# Autodesk Inventor assembly: Intake&Outake
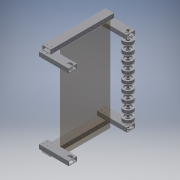
[picture p0: Inventor's stored thumbnail of the model, 180x180]
Saved by Autodesk Inventor 2018 (Build 220112000, 112)
## iProperties
Created: 2018-09-06
Part Number: Intake&Outake
Document SubType Name: Assembly
Designer: baoan
Author: baoan
## Documents named in this file (7)
- C:\Users\baoan\Documents\Inventor\Bunnybots\Intake&Outake\Intake&Outake.iam
- C:\Users\baoan\Documents\Inventor\Bunnybots\Intake&Outake\Vertical_intake_frame.ipt
- C:\Users\baoan\Documents\Inventor\Bunnybots\Intake&Outake\Horizontal_intake_hanger.ipt
- C:\Users\baoan\Documents\Inventor\Bunnybots\Intake&Outake\Bearing.ipt
- C:\Users\baoan\Documents\Inventor\Bunnybots\Intake&Outake\Hex_shaft.ipt
- C:\Users\baoan\Documents\Inventor\Bunnybots\Intake&Outake\36t_x_15mm_Wide_Aluminum_Pulley_HTD_5mm_1_2_Hex_217-4103.ipt
- C:\Users\baoan\Documents\Inventor\Bunnybots\Intake&Outake\Intake_backboard.ipt
## Components (21 placed, 6 different names)
1. Vertical_intake_frame:1 — Flush:1, Mate:1, Flush:2, Flush:5, Flush:6, Mate:3, Mate:19, Flush:14, Flush:16, Mate:20, Flush:17
2. Horizontal_intake_hanger:1 — Flush:1, Mate:1, Flush:2, Insert:7, Insert:8, Mate:21
3. Vertical_intake_frame:2 — Mate:2, Flush:3, Flush:4, Flush:5, Flush:6, Mate:3, Mate:17, Flush:13
4. Horizontal_intake_hanger:2 — Mate:2, Flush:3, Flush:4, Insert:5, Insert:6, Flush:12, Mate:16
5. Bearing:5 — Insert:6, Mate:14
6. Bearing:6 — Insert:5
7. Bearing:7 — Insert:7
8. Bearing:8 — Insert:8
9. Hex_shaft:2 — Flush:12, Angle:1
10. Horizontal_intake_hanger:3 — Mate:17, Flush:13, Flush:15
11. Horizontal_intake_hanger:4 — Mate:19, Flush:14, Flush:15, Flush:16
12. Intake_backboard:1 — Mate:20, Flush:17, Mate:21
13. 36t_x_15mm_Wide_Aluminum_Pulley_HTD_5mm_1_2_Hex_217-4103:1 — Mate:14, Angle:1, Mate:16
14. 36t_x_15mm_Wide_Aluminum_Pulley_HTD_5mm_1_2_Hex_217-4103:2
15. 36t_x_15mm_Wide_Aluminum_Pulley_HTD_5mm_1_2_Hex_217-4103:3
16. 36t_x_15mm_Wide_Aluminum_Pulley_HTD_5mm_1_2_Hex_217-4103:4
17. 36t_x_15mm_Wide_Aluminum_Pulley_HTD_5mm_1_2_Hex_217-4103:5
18. 36t_x_15mm_Wide_Aluminum_Pulley_HTD_5mm_1_2_Hex_217-4103:6
19. 36t_x_15mm_Wide_Aluminum_Pulley_HTD_5mm_1_2_Hex_217-4103:7
20. 36t_x_15mm_Wide_Aluminum_Pulley_HTD_5mm_1_2_Hex_217-4103:8
21. 36t_x_15mm_Wide_Aluminum_Pulley_HTD_5mm_1_2_Hex_217-4103:9
## Component patterns: (9 elements, first: 36t_x_15mm_Wide_Aluminum_Pulley_HTD_5mm_1_2_Hex_217-4103:1)
## Relationships (30: Flush 14, Mate 11, Insert 4, Angle 1)
- Flush:1: Vertical_intake_frame:1 ↔ Horizontal_intake_hanger:1
- Mate:1: Vertical_intake_frame:1 ↔ Horizontal_intake_hanger:1
- Flush:2: Vertical_intake_frame:1 ↔ Horizontal_intake_hanger:1
- Mate:2: Vertical_intake_frame:2 ↔ Horizontal_intake_hanger:2
- Flush:3: Vertical_intake_frame:2 ↔ Horizontal_intake_hanger:2
- Flush:4: Vertical_intake_frame:2 ↔ Horizontal_intake_hanger:2
- Flush:5: Vertical_intake_frame:1 ↔ Vertical_intake_frame:2
- Flush:6: Vertical_intake_frame:1 ↔ Vertical_intake_frame:2
- Mate:3 (508 mm): Vertical_intake_frame:1 ↔ Vertical_intake_frame:2
- [Flush]: Bearing:5 ↔ Bearing:6
- [Flush]: Bearing:7 ↔ Bearing:8
- [Mate]: Bearing:6 ↔ Hex_shaft:2
- [Mate]: Bearing:6 ↔ Hex_shaft:2
- Insert:5: Horizontal_intake_hanger:2 ↔ Bearing:6
- Insert:6: Horizontal_intake_hanger:2 ↔ Bearing:5
- Insert:7: Horizontal_intake_hanger:1 ↔ Bearing:7
- Insert:8: Horizontal_intake_hanger:1 ↔ Bearing:8
- Flush:12 (-12.7 mm): Horizontal_intake_hanger:2 ↔ Hex_shaft:2
- Mate:14: Bearing:5 ↔ 36t_x_15mm_Wide_Aluminum_Pulley_HTD_5mm_1_2_Hex_217-4103:1
- Angle:1 (0 deg): Hex_shaft:2 ↔ 36t_x_15mm_Wide_Aluminum_Pulley_HTD_5mm_1_2_Hex_217-4103:1
- Mate:16 (12.7 mm): Horizontal_intake_hanger:2 ↔ 36t_x_15mm_Wide_Aluminum_Pulley_HTD_5mm_1_2_Hex_217-4103:1
- Mate:17: Vertical_intake_frame:2 ↔ Horizontal_intake_hanger:3
- Flush:13: Vertical_intake_frame:2 ↔ Horizontal_intake_hanger:3
- Mate:19: Vertical_intake_frame:1 ↔ Horizontal_intake_hanger:4
- Flush:14: Vertical_intake_frame:1 ↔ Horizontal_intake_hanger:4
- Flush:15: Horizontal_intake_hanger:3 ↔ Horizontal_intake_hanger:4
- Flush:16 (-19.05 mm): Vertical_intake_frame:1 ↔ Horizontal_intake_hanger:4
- Mate:20 (25.4 mm): Vertical_intake_frame:1 ↔ Intake_backboard:1
- Flush:17: Vertical_intake_frame:1 ↔ Intake_backboard:1
- Mate:21: Horizontal_intake_hanger:1 ↔ Intake_backboard:1
## Named parameters: d37_d31 = 0 mm, d38_d32 = 0 mm, d39_d34 = 0 mm, d40_d35 = 0 mm
